# Autodesk Inventor assembly: Rad_Schutz
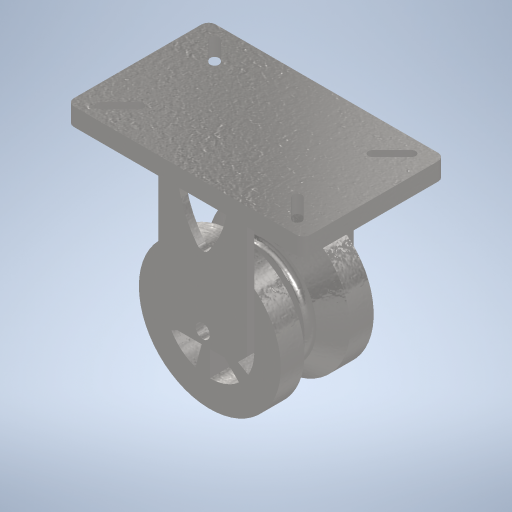
[picture p0: Inventor's stored thumbnail of the model, 512x512]
Saved by Autodesk Inventor 2024 (Build 280153000, 153)
## iProperties
Created: 2024-02-12
Part Number: Rad_Schutz
Document SubType Name: Assembly
Designer: ffogue
Author: ffogue
## Documents named in this file (3)
- C:\Users\ffogue\OneDrive - MuM - OM\Dokumente\Inventor\Motor\Rad_Schutz.iam
- C:\Users\ffogue\OneDrive - MuM - OM\Dokumente\Inventor\Motor\Koerper.ipt
- C:\Users\ffogue\OneDrive - MuM - OM\Dokumente\Inventor\Motor\Rad.ipt
## Components (2 placed, 2 different names)
1. Koerper:1 — Passend:1
2. Rad:1 — Passend:1
## Relationships (1: Mate 1)
- Passend:1 [Mate]: Koerper:1 ↔ Rad:1
